# Autodesk Inventor assembly: coxa kanan
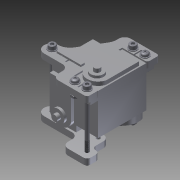
[picture p0: Inventor's stored thumbnail of the model, 180x180]
Saved by Autodesk Inventor 2012 (Build 160160000, 160)
## iProperties
Created: 2013-12-07
Part Number: coxa kanan
Document SubType Name: Assembly
Designer: Irwan Haryanto
Author: Irwan Haryanto
## Documents named in this file (9)
- D:\Revenant\robot baru 2014\coxa kanan.iam
- D:\Revenant\robot baru 2014\braket atas.ipt
- D:\Revenant\robot baru 2014\braket bawah.ipt
- D:\Revenant\robot baru 2014\servo HS-7955GT.ipt
- D:\Revenant\robot baru 2014\coxa kanan\Design Accelerator\Bolted Connection1.iam
- D:\Revenant\robot baru 2014\coxa kanan\Design Accelerator\Bolted Connection2.iam
- D:\Revenant\robot baru 2014\coxa kanan\Design Accelerator\Bolted Connection3.iam
- D:\Revenant\robot baru 2014\coxa kanan\Design Accelerator\Bolted Connection4.iam
- D:\Revenant\robot baru 2014\coxa kanan\Design Accelerator\Bolted Connection5.iam
## Components (9 placed, 4 different names)
1. braket atas:1 — Mate:1, Mate:2, Mate:3, Insert:1, Insert:2, Mate:20, Mate:22, Mate:24, Mate:26, Mate:28, Insert:3, Insert:4
2. braket bawah:1 — Mate:4, Mate:5, Mate:6, Mate:7, Mate:25, Mate:27, Mate:29
3. servo HS-7955GT:1 — Mate:1, Mate:2, Mate:3, Mate:4, Mate:5, Mate:6, Mate:7
4. Bolted Connection:1 [sub-assembly] — Mate:24, Mate:25
5. Bolted Connection:2 [sub-assembly] — Mate:26, Mate:27
6. Bolted Connection:3 [sub-assembly] — Mate:28, Mate:29
7. servo HS-7955GT:2 — Insert:1, Insert:2, Mate:21, Mate:23, Insert:3, Insert:4
8. Bolted Connection:4 [sub-assembly] — Mate:20, Mate:21
9. Bolted Connection:5 [sub-assembly] — Mate:22, Mate:23
## Relationships (21: Mate 17, Insert 4)
- Mate:1: braket atas:1 ↔ servo HS-7955GT:1
- Mate:2: braket atas:1 ↔ servo HS-7955GT:1
- Mate:3: braket atas:1 ↔ servo HS-7955GT:1
- Mate:4: braket bawah:1 ↔ servo HS-7955GT:1
- Mate:5: braket bawah:1 ↔ servo HS-7955GT:1
- Mate:6: braket bawah:1 ↔ servo HS-7955GT:1
- Mate:7: braket bawah:1 ↔ servo HS-7955GT:1
- Insert:1: braket atas:1 ↔ servo HS-7955GT:2
- Insert:2: braket atas:1 ↔ servo HS-7955GT:2
- Mate:20: braket atas:1 ↔ Bolted Connection:4
- Mate:21: servo HS-7955GT:2 ↔ Bolted Connection:4
- Mate:22: braket atas:1 ↔ Bolted Connection:5
- Mate:23: servo HS-7955GT:2 ↔ Bolted Connection:5
- Mate:24: braket atas:1 ↔ Bolted Connection:1
- Mate:25: braket bawah:1 ↔ Bolted Connection:1
- Mate:26: braket atas:1 ↔ Bolted Connection:2
- Mate:27: braket bawah:1 ↔ Bolted Connection:2
- Mate:28: braket atas:1 ↔ Bolted Connection:3
- Mate:29: braket bawah:1 ↔ Bolted Connection:3
- Insert:3: braket atas:1 ↔ servo HS-7955GT:2
- Insert:4: braket atas:1 ↔ servo HS-7955GT:2
